# Autodesk Inventor assembly: Sestava
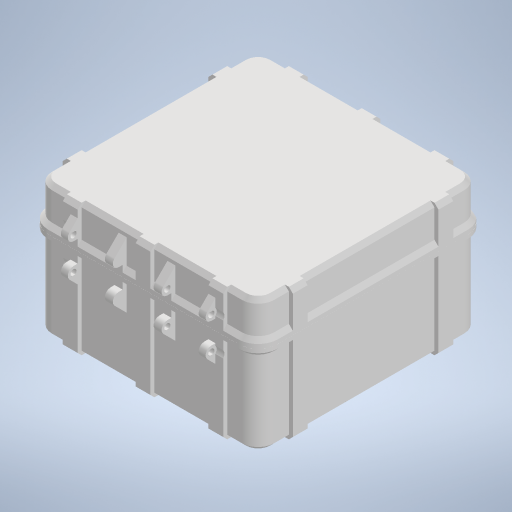
[picture p0: Inventor's stored thumbnail of the model, 512x512]
Saved by Autodesk Inventor 2024 (Build 280153000, 153)
## iProperties
Created: 2024-03-05
Part Number: Sestava
Document SubType Name: Assembly
Designer: Simak
Author: Simak
## Documents named in this file (6)
- C:\Users\42060\Desktop\Sumec krabička\Sestava.iam
- C:\Users\42060\Desktop\Sumec krabička\universal_box-lid.ipt
- C:\Users\42060\Desktop\Sumec krabička\universal_box-main_body.ipt
- C:\Users\42060\Desktop\Sumec krabička\horni_vlozka.ipt
- C:\Users\42060\Desktop\Sumec krabička\spodni_vlozka.ipt
- C:\Users\42060\Desktop\ŠKOLA\Mini sumo\RoboCop\- 3D -\_wip\Sestava.iam
## Components (5 placed, 5 different names)
1. universal_box-lid:1 — Stejný směr:1, Proti sobě:1, Proti sobě:2, Vložit:1, Proti sobě:6, Proti sobě:7, Proti sobě:8
2. universal_box-main_body:1 — Stejný směr:1, Proti sobě:1, Proti sobě:2, Vložit:1, Proti sobě:3, Proti sobě:4, Proti sobě:5
3. horni_vlozka:1 — Proti sobě:6, Proti sobě:7, Proti sobě:8
4. spodni_vlozka:1 — Proti sobě:3, Proti sobě:4, Proti sobě:5, Proti sobě:9, Proti sobě:10
5. Sestava:1 [sub-assembly] — Proti sobě:9, Proti sobě:10
## Relationships (12: Mate 10, Flush 1, Insert 1)
- Stejný směr:1 [Flush]: universal_box-lid:1 ↔ universal_box-main_body:1
- Proti sobě:1 [Mate]: universal_box-lid:1 ↔ universal_box-main_body:1
- Proti sobě:2 [Mate]: universal_box-lid:1 ↔ universal_box-main_body:1
- Vložit:1 [Insert]: universal_box-lid:1 ↔ universal_box-main_body:1
- Proti sobě:3 [Mate]: universal_box-main_body:1 ↔ spodni_vlozka:1
- Proti sobě:4 [Mate]: universal_box-main_body:1 ↔ spodni_vlozka:1
- Proti sobě:5 [Mate]: universal_box-main_body:1 ↔ spodni_vlozka:1
- Proti sobě:6 [Mate]: universal_box-lid:1 ↔ horni_vlozka:1
- Proti sobě:7 [Mate]: universal_box-lid:1 ↔ horni_vlozka:1
- Proti sobě:8 [Mate]: universal_box-lid:1 ↔ horni_vlozka:1
- Proti sobě:9 [Mate]: spodni_vlozka:1 ↔ Sestava:1
- Proti sobě:10 [Mate] (-0.25 mm): spodni_vlozka:1 ↔ Sestava:1
